# Autodesk Inventor assembly: Soyuz Fairing & Payload Bay Assembly Grid Fin Deploy
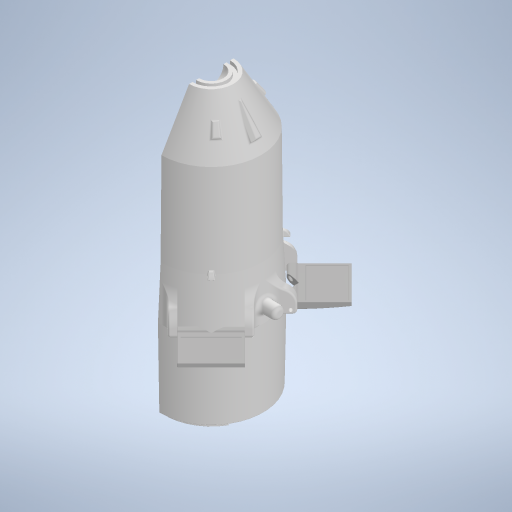
[picture p0: Inventor's stored thumbnail of the model, 512x512]
Saved by Autodesk Inventor 2023 (Build 270158030, 158C)
## iProperties
Created: 2023-01-09
Part Number: Soyuz Fairing & Payload Bay Assembly Grid Fin Deploy
Document SubType Name: Assembly
Designer: Imogen Heard
Author: Imogen Heard
## Documents named in this file (3)
- C:\Users\dheard\Documents\Inventor\Inventor_Projects\Soyuz Model\Soyuz Fairing & Payload Bay Assembly Grid Fin Deploy.iam
- C:\Users\dheard\Documents\Inventor\Inventor_Projects\Soyuz Model\Fairing.ipt
- C:\Users\dheard\Documents\Inventor\Inventor_Projects\Soyuz Model\Grid Fins.ipt
## Components (3 placed, 2 different names)
1. Fairing:1 — Rotational:1, Rotational:2
2. Grid Fins:1 — Rotational:1
3. Grid Fins:2 — Rotational:2
## Relationships (2: RevoluteJoint 2)
- Rotational:1 [RevoluteJoint]: Fairing:1 ↔ Grid Fins:1
- Rotational:2 [RevoluteJoint]: Fairing:1 ↔ Grid Fins:2
